# Autodesk Inventor assembly: Transmisión de correa trapezoidal
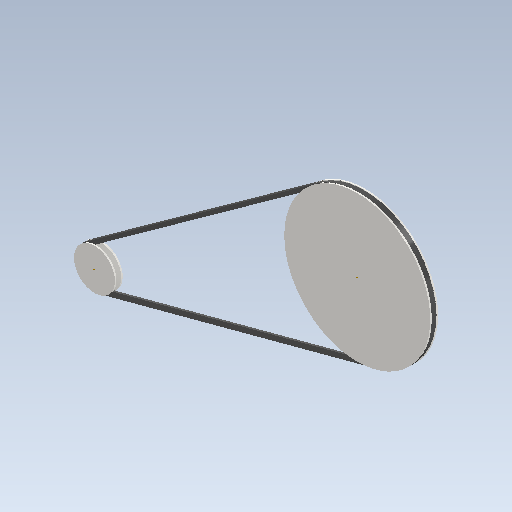
[picture p0: Inventor's stored thumbnail of the model, 512x512]
Saved by Autodesk Inventor 2020.5 (Build 245400000, 400)
## iProperties
ClientObjectVersion: 1
Created: 2022-12-03
Part Number: Transmisión de correa trapezoidal
Document SubType Name: Assembly
Designer: André Aguirre Apolo
Author: André Aguirre Apolo
## Documents named in this file (4)
- C:\Users\André Aguirre Apolo\Desktop\ESPOL\PAO2, 2022\Diseño y simulacion de maquinas\Teorico\Tarea2\Ensamblaje1\Design Accelerator\Transmisión de correa trapezoidal2.iam
- C:\Users\André Aguirre Apolo\Desktop\ESPOL\PAO2, 2022\Diseño y simulacion de maquinas\Teorico\Tarea2\Ensamblaje1\Design Accelerator\Correa trapezoidal2.ipt
- C:\Users\André Aguirre Apolo\Desktop\ESPOL\PAO2, 2022\Diseño y simulacion de maquinas\Teorico\Tarea2\Ensamblaje1\Design Accelerator\Polea ranurada12.ipt
- C:\Users\André Aguirre Apolo\Desktop\ESPOL\PAO2, 2022\Diseño y simulacion de maquinas\Teorico\Tarea2\Ensamblaje1\Design Accelerator\Polea ranurada22.ipt
## Components (3 placed, 3 different names)
1. Polea ranurada1:1 — Nivelación:1, Coincidencia:1, Rotación:1
2. Polea ranurada2:1 — Nivelación:2, Coincidencia:2, Rotación:1
3. Correa trapezoidal:1 — Nivelación:1, Coincidencia:1, Nivelación:2, Coincidencia:2
## Component patterns: (1 elements, first: Correa trapezoidal:1)
## Relationships (5: Flush 2, Mate 2, RelateRotation 1)
- Nivelación:1 [Flush]: Polea ranurada1:1 ↔ Correa trapezoidal:1
- Coincidencia:1 [Mate]: Polea ranurada1:1 ↔ Correa trapezoidal:1
- Nivelación:2 [Flush]: Polea ranurada2:1 ↔ Correa trapezoidal:1
- Coincidencia:2 [Mate]: Polea ranurada2:1 ↔ Correa trapezoidal:1
- Rotación:1 [RelateRotation] (3.6875 ul): Polea ranurada1:1 ↔ Polea ranurada2:1
